# Autodesk Inventor assembly: OPTICS FOCUS MOZ-200-25
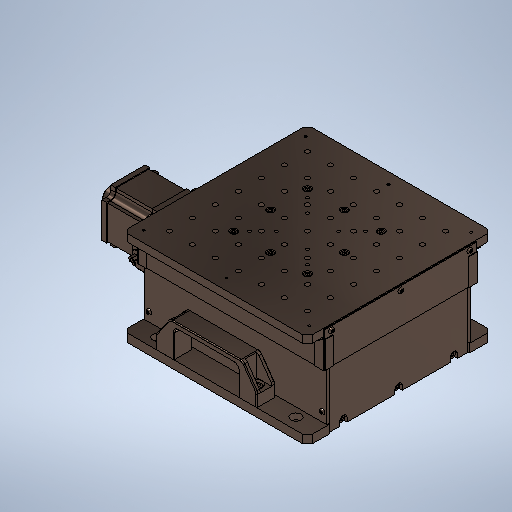
[picture p0: Inventor's stored thumbnail of the model, 512x512]
Saved by Autodesk Inventor 2025.3 (Build 293356000, 356)
## iProperties
RuleStatus: InUse
AfterDocSave0: file://Part Number Cleaner
Created: 2019-09-04
Vendor: HHMI: JRC - ID&F
Document SubType Name: Assembly
Designer: arnoldj
DESIGN DEPARTMENT: HHMI: JRC - ID&F
ALTERED ITEM PART NUMBER: N/A
ALTERED ITEM VENDOR: N/A
ALTERED ITEM DESCRIPTION: N/A
Author: arnoldj
Revision Number: 0
## Documents named in this file (3)
- C:\_WORKSPACE\DATA\COMMON\Optics Focus\OPTICS FOCUS MOZ-200-25.iam
- C:\_WORKSPACE\DATA\COMMON\Optics Focus\OPTICS FOCUS MOZ-200-25_BASE.ipt
- C:\_WORKSPACE\DATA\COMMON\Optics Focus\OPTICS FOCUS_MOZ-200-25_CARR.ipt
## Components (2 placed, 2 different names)
1. OPTICS FOCUS MOZ-200-25_BASE:1 — Flush:1, Flush:2, Mate:1
2. OPTICS FOCUS_MOZ-200-25_CARR:1 — Flush:1, Flush:2, Mate:1
## Relationships (3: Flush 2, Mate 1)
- Flush:1: OPTICS FOCUS MOZ-200-25_BASE:1 ↔ OPTICS FOCUS_MOZ-200-25_CARR:1
- Flush:2: OPTICS FOCUS MOZ-200-25_BASE:1 ↔ OPTICS FOCUS_MOZ-200-25_CARR:1
- Mate:1 (102.5 mm): OPTICS FOCUS MOZ-200-25_BASE:1 ↔ OPTICS FOCUS_MOZ-200-25_CARR:1
